# Autodesk Inventor assembly: сборка системы полива норм
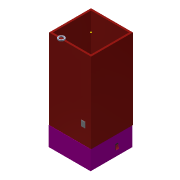
[picture p0: Inventor's stored thumbnail of the model, 180x180]
Saved by Autodesk Inventor 2022 (Build 260153000, 153)
## iProperties
Created: 2023-02-10
Part Number: сборка системы полива норм
Document SubType Name: Assembly
Designer: Egori
Mass: 957.74 g
Surface Area: 2859.39 cm^2
Volume: 822.826 cm^3
Density: 1.16396 g/cm^3
Author: Egori
## Documents named in this file (6)
- C:\Теплица\сборка системы полива норм.iam
- C:\Теплица\баллон с водой.ipt
- C:\Теплица\датчик уровня водыtouch button TTP223.ipt
- C:\Теплица\насос погружной.ipt
- C:\Теплица\sponge.ipt
- C:\Теплица\сборка с коробочкой для системы полива.iam
## Components (5 placed, 5 different names)
1. баллон с водой:1 — Жесткий:1, Совмещение:1, Совмещение:2, Совмещение:3
2. датчик уровня водыtouch button TTP223:1 — Совмещение:1
3. насос погружной:1 — Жесткий:1
4. ультразвуковой увлажниьель воздуха — Совмещение:2
5. сборка с коробочкой для системы полива:1 [sub-assembly] — Совмещение:3
## Relationships (4: Mate 3, WeldJoint 1)
- Жесткий:1 [WeldJoint]: баллон с водой:1 ↔ насос погружной:1
- Совмещение:1 [Mate]: баллон с водой:1 ↔ датчик уровня водыtouch button TTP223:1
- Совмещение:2 [Mate]: баллон с водой:1 ↔ ультразвуковой увлажниьель воздуха
- Совмещение:3 [Mate]: баллон с водой:1 ↔ сборка с коробочкой для системы полива:1
